# Autodesk Inventor assembly: Backhoe
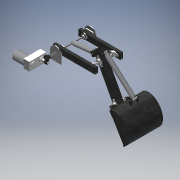
[picture p0: Inventor's stored thumbnail of the model, 180x180]
Saved by Autodesk Inventor 2019 (Build 230136000, 136)
## iProperties
Created: 2018-10-28
Part Number: Backhoe
Document SubType Name: Assembly
Designer: Alex Barnett
Mass: 10369.2 g
Surface Area: 11607 cm^2
Volume: 2447.16 cm^3
Density: 4.23725 g/cm^3
Author: Alex Barnett
## Documents named in this file (21)
- C:\Users\Alex Barnett\Documents\Machine Design\PR2\CAD\Backhoe.iam
- C:\Users\Alex Barnett\Documents\Machine Design\PR2\CAD\Boom Hinge.ipt
- C:\Users\Alex Barnett\Documents\Machine Design\PR2\CAD\Pin .5in. Dia. - Boom Hinge.ipt
- C:\Users\Alex Barnett\Documents\Machine Design\PR2\CAD\Steel 4130 1x2in. Tubing, t=.065in.,L=15in..ipt
- C:\Users\Alex Barnett\Documents\Machine Design\PR2\CAD\Steel 4130 1x2in. Tubing, t=.065in.,L=22in..ipt
- C:\Users\Alex Barnett\Documents\Machine Design\PR2\CAD\Boom to Stick .5in. Pin.ipt
- C:\Users\Alex Barnett\Documents\Machine Design\PR2\CAD\AmpFlow Motor & Gearbox.iam
- C:\Users\Alex Barnett\Documents\Machine Design\PR2\CAD\Worm Gear 12P 18T.ipt
- C:\Users\Alex Barnett\Documents\Machine Design\PR2\CAD\Steel 4130 1x2in. Tubing, t=.065in.,L=22in. Mirrored.ipt
- C:\Users\Alex Barnett\Documents\Machine Design\PR2\CAD\Stick to Scoop .5in. Pin.ipt
- C:\Users\Alex Barnett\Documents\Machine Design\PR2\CAD\Bucket.ipt
- C:\Users\Alex Barnett\Documents\Machine Design\PR2\CAD\Linear Actuator Top Pin .5in. Dia..ipt
- C:\Users\Alex Barnett\Documents\Machine Design\PR2\CAD\Linear Actuator Top Scoop Pin .5in. Dia..ipt
- C:\Users\Alex Barnett\Documents\Machine Design\PR2\CAD\Dry-Running Two-Bolt Flange Mounted Bearing, 0.5in. Diameter.ipt
- C:\Users\Alex Barnett\Documents\Machine Design\PR2\CAD\External Retaining Ring - Stainless Steel. 0.5in. Diameter.ipt
- C:\Users\Alex Barnett\Documents\Machine Design\PR2\CAD\Hub Connected to Steel Tubing - 0.5in. Diameter.ipt
- C:\Users\Alex Barnett\Documents\Machine Design\PR2\CAD\Tapered Roller Bearing Housing.ipt
- C:\Users\Alex Barnett\Documents\Machine Design\PR2\CAD\Tapered Roller Bearing, 0.5in. Diameter.ipt
- C:\Users\Alex Barnett\Documents\Machine Design\PR2\CAD\.125in. X .125in. Key, 1in. Long.ipt
- C:\Users\Alex Barnett\Documents\Machine Design\PR2\CAD\7.5 inch Linear Actuator.ipt
- C:\Users\Alex Barnett\Documents\Machine Design\PR2\CAD\9 inch Linear Actuator.ipt
## Components (45 placed, 20 different names)
1. Boom Hinge:1 — Mate:1, Mate:2, Mate:3, Flush:2, Mate:6, Mate:131, Mate:142, Mate:144, Mate:145, Mate:164
2. Boom Hinge:2 — Mate:5, Flush:2, Flush:5, Flush:11, Mate:129, Mate:147, Mate:149, Mate:150
3. Pin .5in. Dia. - Boom Hinge:1 — Mate:5, Mate:6, Flush:5, Mate:21, Mate:67, Mate:68, Mate:136, Mate:137, Mate:138, Mate:139, Mate:141, Mate:143, Mate:146, Mate:148, Mate:151, Mate:154, Flush:23, Mate:156, Mate:159, Mate:160, Mate:163, Mate:197
4. Steel 4130 1x2in. Tubing, t=.065in.,L=15in.:1 — Flush:6, Mate:21, Mate:110, Mate:112, Mate:113, Mate:130, Mate:131, Mate:140, Mate:152, Mate:158
5. Steel 4130 1x2in. Tubing, t=.065in.,L=15in.:2 — Flush:6, Mate:114, Mate:116, Mate:129, Mate:130, Mate:153, Mate:161, Mate:162, Mate:164
6. Boom to Stick .5in. Pin:1 — Mate:72, Mate:73, Mate:80, Mate:111, Mate:113, Mate:115, Mate:118, Mate:121, Mate:166, Mate:168, Mate:189, Mate:190, Mate:192
7. AmpFlow Motor & Gearbox:1 [sub-assembly] — Mate:69, Mate:70, Mate:71
8. Worm Gear 12P 18T:1 — Mate:67, Mate:68, Mate:69, Mate:70, Mate:71
9. Steel 4130 1x2in. Tubing, t=.065in.,L=22in.:1 — Mate:72, Mate:73, Flush:17, Mate:84, Mate:95, Mate:117, Mate:119, Mate:123, Mate:124, Mate:125, Mate:183, Mate:187
10. Steel 4130 1x2in. Tubing, t=.065in.,L=22in. Mirrored:1 — Mate:80, Flush:17, Mate:84, Flush:18, Mate:91, Flush:21, Flush:22, Mate:103, Mate:120, Mate:122, Mate:126, Mate:127, Mate:128, Mate:163, Mate:181, Mate:185
11. Stick to Scoop .5in. Pin:1 — Flush:18, Mate:169, Mate:170, Mate:174, Mate:176
12. Bucket:1 — Mate:170, Flush:24, Mate:171, Mate:172, Mate:173, Mate:175, Mate:177, Mate:179
13. Linear Actuator Top Pin .5in. Dia.:1 — Mate:91, Flush:21, Mate:182, Mate:184, Mate:199
14. Linear Actuator Top Scoop Pin .5in. Dia.:1 — Mate:171, Mate:172, Mate:178, Mate:180, Mate:200
15. Linear Actuator Top Pin .5in. Dia.:2 — Mate:95, Flush:22, Mate:186, Mate:188, Mate:198
16. Dry-Running Two-Bolt Flange Mounted Bearing, 0.5in. Diameter:5 — Mate:110, Mate:111, Mate:112, Mate:167
17. Dry-Running Two-Bolt Flange Mounted Bearing, 0.5in. Diameter:6 — Mate:114, Mate:115, Mate:116, Mate:165
18. Dry-Running Two-Bolt Flange Mounted Bearing, 0.5in. Diameter:7 — Mate:117, Mate:118, Mate:119, Mate:191
19. Dry-Running Two-Bolt Flange Mounted Bearing, 0.5in. Diameter:8 — Mate:120, Mate:121, Mate:122
20. Dry-Running Two-Bolt Flange Mounted Bearing, 0.5in. Diameter:9 — Mate:123, Mate:124, Mate:125, Mate:169
21. Dry-Running Two-Bolt Flange Mounted Bearing, 0.5in. Diameter:10 — Mate:126, Mate:127, Mate:128
22. External Retaining Ring - Stainless Steel. 0.5in. Diameter:1 — Mate:136, Mate:137
23. External Retaining Ring - Stainless Steel. 0.5in. Diameter:2 — Mate:138, Mate:139
24. Hub Connected to Steel Tubing - 0.5in. Diameter:1 — Mate:140, Mate:141, Mate:152, Flush:23, Mate:157
25. Tapered Roller Bearing Housing:1 — Mate:142, Mate:143, Mate:144
26. Tapered Roller Bearing, 0.5in. Diameter:1 — Mate:145, Mate:146
27. Tapered Roller Bearing Housing:2 — Mate:147, Mate:148, Mate:149
28. Tapered Roller Bearing, 0.5in. Diameter:2 — Mate:150, Mate:151
29. Hub Connected to Steel Tubing - 0.5in. Diameter:2 — Mate:153, Mate:154, Mate:161
30. .125in. X .125in. Key, 1in. Long:1 — Mate:156, Mate:157, Mate:158
31. .125in. X .125in. Key, 1in. Long:2 — Mate:159, Mate:160, Mate:162
32. External Retaining Ring - Stainless Steel. 0.5in. Diameter:3 — Mate:165, Mate:166
33. External Retaining Ring - Stainless Steel. 0.5in. Diameter:4 — Mate:167, Mate:168
34. External Retaining Ring - Stainless Steel. 0.5in. Diameter:5 — Mate:173, Mate:174
35. External Retaining Ring - Stainless Steel. 0.5in. Diameter:6 — Mate:175, Mate:176
36. External Retaining Ring - Stainless Steel. 0.5in. Diameter:7 — Mate:177, Mate:178
37. External Retaining Ring - Stainless Steel. 0.5in. Diameter:8 — Mate:179, Mate:180
38. External Retaining Ring - Stainless Steel. 0.5in. Diameter:9 — Mate:181, Mate:182
39. External Retaining Ring - Stainless Steel. 0.5in. Diameter:10 — Mate:183, Mate:184
40. External Retaining Ring - Stainless Steel. 0.5in. Diameter:11 — Mate:185, Mate:186
41. External Retaining Ring - Stainless Steel. 0.5in. Diameter:12 — Mate:187, Mate:188
42. External Retaining Ring - Stainless Steel. 0.5in. Diameter:13 — Mate:189, Mate:190
43. External Retaining Ring - Stainless Steel. 0.5in. Diameter:14 — Mate:191, Mate:192
44. 7.5 inch Linear Actuator:1 — Mate:197, Mate:198
45. 9 inch Linear Actuator:1 — Mate:199, Mate:200
## Relationships (112: Mate 100, Flush 12)
- Mate:1: Boom Hinge:1
- Mate:2: Boom Hinge:1
- Mate:3: Boom Hinge:1
- Mate:5: Boom Hinge:2 ↔ Pin .5in. Dia. - Boom Hinge:1
- Flush:2: Boom Hinge:1 ↔ Boom Hinge:2
- Mate:6: Boom Hinge:1 ↔ Pin .5in. Dia. - Boom Hinge:1
- Flush:5: Boom Hinge:2 ↔ Pin .5in. Dia. - Boom Hinge:1
- Flush:6: Steel 4130 1x2in. Tubing, t=.065in.,L=15in.:1 ↔ Steel 4130 1x2in. Tubing, t=.065in.,L=15in.:2
- Mate:21: Pin .5in. Dia. - Boom Hinge:1 ↔ Steel 4130 1x2in. Tubing, t=.065in.,L=15in.:1
- Flush:11: Boom Hinge:2
- Flush:12 (300 mm)
- Flush:13 (500 mm)
- Mate:67: Pin .5in. Dia. - Boom Hinge:1 ↔ Worm Gear 12P 18T:1
- Mate:68: Pin .5in. Dia. - Boom Hinge:1 ↔ Worm Gear 12P 18T:1
- Mate:69: AmpFlow Motor & Gearbox:1 ↔ Worm Gear 12P 18T:1
- Mate:70: AmpFlow Motor & Gearbox:1 ↔ Worm Gear 12P 18T:1
- Mate:71: AmpFlow Motor & Gearbox:1 ↔ Worm Gear 12P 18T:1
- Mate:72: Boom to Stick .5in. Pin:1 ↔ Steel 4130 1x2in. Tubing, t=.065in.,L=22in.:1
- Mate:73: Boom to Stick .5in. Pin:1 ↔ Steel 4130 1x2in. Tubing, t=.065in.,L=22in.:1
- Mate:80: Boom to Stick .5in. Pin:1 ↔ Steel 4130 1x2in. Tubing, t=.065in.,L=22in. Mirrored:1
- Flush:17: Steel 4130 1x2in. Tubing, t=.065in.,L=22in.:1 ↔ Steel 4130 1x2in. Tubing, t=.065in.,L=22in. Mirrored:1
- Mate:84: Steel 4130 1x2in. Tubing, t=.065in.,L=22in.:1 ↔ Steel 4130 1x2in. Tubing, t=.065in.,L=22in. Mirrored:1
- Flush:18: Steel 4130 1x2in. Tubing, t=.065in.,L=22in. Mirrored:1 ↔ Stick to Scoop .5in. Pin:1
- Mate:91: Steel 4130 1x2in. Tubing, t=.065in.,L=22in. Mirrored:1 ↔ Linear Actuator Top Pin .5in. Dia.:1
- Flush:21: Steel 4130 1x2in. Tubing, t=.065in.,L=22in. Mirrored:1 ↔ Linear Actuator Top Pin .5in. Dia.:1
- Mate:95: Steel 4130 1x2in. Tubing, t=.065in.,L=22in.:1 ↔ Linear Actuator Top Pin .5in. Dia.:2
- Flush:22: Steel 4130 1x2in. Tubing, t=.065in.,L=22in. Mirrored:1 ↔ Linear Actuator Top Pin .5in. Dia.:2
- Mate:103: Steel 4130 1x2in. Tubing, t=.065in.,L=22in. Mirrored:1
- Mate:110: Steel 4130 1x2in. Tubing, t=.065in.,L=15in.:1 ↔ Dry-Running Two-Bolt Flange Mounted Bearing, 0.5in. Diameter:5
- Mate:111: Boom to Stick .5in. Pin:1 ↔ Dry-Running Two-Bolt Flange Mounted Bearing, 0.5in. Diameter:5
- Mate:112: Steel 4130 1x2in. Tubing, t=.065in.,L=15in.:1 ↔ Dry-Running Two-Bolt Flange Mounted Bearing, 0.5in. Diameter:5
- Mate:113: Steel 4130 1x2in. Tubing, t=.065in.,L=15in.:1 ↔ Boom to Stick .5in. Pin:1
- Mate:114: Steel 4130 1x2in. Tubing, t=.065in.,L=15in.:2 ↔ Dry-Running Two-Bolt Flange Mounted Bearing, 0.5in. Diameter:6
- Mate:115: Boom to Stick .5in. Pin:1 ↔ Dry-Running Two-Bolt Flange Mounted Bearing, 0.5in. Diameter:6
- Mate:116: Steel 4130 1x2in. Tubing, t=.065in.,L=15in.:2 ↔ Dry-Running Two-Bolt Flange Mounted Bearing, 0.5in. Diameter:6
- Mate:117: Steel 4130 1x2in. Tubing, t=.065in.,L=22in.:1 ↔ Dry-Running Two-Bolt Flange Mounted Bearing, 0.5in. Diameter:7
- Mate:118: Boom to Stick .5in. Pin:1 ↔ Dry-Running Two-Bolt Flange Mounted Bearing, 0.5in. Diameter:7
- Mate:119: Steel 4130 1x2in. Tubing, t=.065in.,L=22in.:1 ↔ Dry-Running Two-Bolt Flange Mounted Bearing, 0.5in. Diameter:7
- Mate:120: Steel 4130 1x2in. Tubing, t=.065in.,L=22in. Mirrored:1 ↔ Dry-Running Two-Bolt Flange Mounted Bearing, 0.5in. Diameter:8
- Mate:121: Boom to Stick .5in. Pin:1 ↔ Dry-Running Two-Bolt Flange Mounted Bearing, 0.5in. Diameter:8
- Mate:122: Steel 4130 1x2in. Tubing, t=.065in.,L=22in. Mirrored:1 ↔ Dry-Running Two-Bolt Flange Mounted Bearing, 0.5in. Diameter:8
- Mate:123: Steel 4130 1x2in. Tubing, t=.065in.,L=22in.:1 ↔ Dry-Running Two-Bolt Flange Mounted Bearing, 0.5in. Diameter:9
- Mate:124: Steel 4130 1x2in. Tubing, t=.065in.,L=22in.:1 ↔ Dry-Running Two-Bolt Flange Mounted Bearing, 0.5in. Diameter:9
- Mate:125: Steel 4130 1x2in. Tubing, t=.065in.,L=22in.:1 ↔ Dry-Running Two-Bolt Flange Mounted Bearing, 0.5in. Diameter:9
- Mate:126: Steel 4130 1x2in. Tubing, t=.065in.,L=22in. Mirrored:1 ↔ Dry-Running Two-Bolt Flange Mounted Bearing, 0.5in. Diameter:10
- Mate:127: Steel 4130 1x2in. Tubing, t=.065in.,L=22in. Mirrored:1 ↔ Dry-Running Two-Bolt Flange Mounted Bearing, 0.5in. Diameter:10
- Mate:128: Steel 4130 1x2in. Tubing, t=.065in.,L=22in. Mirrored:1 ↔ Dry-Running Two-Bolt Flange Mounted Bearing, 0.5in. Diameter:10
- Mate:129 (25.4 mm): Boom Hinge:2 ↔ Steel 4130 1x2in. Tubing, t=.065in.,L=15in.:2
- Mate:130 (-254 mm): Steel 4130 1x2in. Tubing, t=.065in.,L=15in.:1 ↔ Steel 4130 1x2in. Tubing, t=.065in.,L=15in.:2
- Mate:131 (25.4 mm): Boom Hinge:1 ↔ Steel 4130 1x2in. Tubing, t=.065in.,L=15in.:1
- Mate:136: Pin .5in. Dia. - Boom Hinge:1 ↔ External Retaining Ring - Stainless Steel. 0.5in. Diameter:1
- Mate:137: Pin .5in. Dia. - Boom Hinge:1 ↔ External Retaining Ring - Stainless Steel. 0.5in. Diameter:1
- Mate:138: Pin .5in. Dia. - Boom Hinge:1 ↔ External Retaining Ring - Stainless Steel. 0.5in. Diameter:2
- Mate:139: Pin .5in. Dia. - Boom Hinge:1 ↔ External Retaining Ring - Stainless Steel. 0.5in. Diameter:2
- Mate:140: Steel 4130 1x2in. Tubing, t=.065in.,L=15in.:1 ↔ Hub Connected to Steel Tubing - 0.5in. Diameter:1
- Mate:141: Pin .5in. Dia. - Boom Hinge:1 ↔ Hub Connected to Steel Tubing - 0.5in. Diameter:1
- Mate:142: Boom Hinge:1 ↔ Tapered Roller Bearing Housing:1
- Mate:143: Pin .5in. Dia. - Boom Hinge:1 ↔ Tapered Roller Bearing Housing:1
- Mate:144: Boom Hinge:1 ↔ Tapered Roller Bearing Housing:1
- Mate:145: Boom Hinge:1 ↔ Tapered Roller Bearing, 0.5in. Diameter:1
- Mate:146: Pin .5in. Dia. - Boom Hinge:1 ↔ Tapered Roller Bearing, 0.5in. Diameter:1
- Mate:147: Boom Hinge:2 ↔ Tapered Roller Bearing Housing:2
- Mate:148: Pin .5in. Dia. - Boom Hinge:1 ↔ Tapered Roller Bearing Housing:2
- Mate:149: Boom Hinge:2 ↔ Tapered Roller Bearing Housing:2
- Mate:150: Boom Hinge:2 ↔ Tapered Roller Bearing, 0.5in. Diameter:2
- Mate:151: Pin .5in. Dia. - Boom Hinge:1 ↔ Tapered Roller Bearing, 0.5in. Diameter:2
- Mate:152: Steel 4130 1x2in. Tubing, t=.065in.,L=15in.:1 ↔ Hub Connected to Steel Tubing - 0.5in. Diameter:1
- Mate:153: Steel 4130 1x2in. Tubing, t=.065in.,L=15in.:2 ↔ Hub Connected to Steel Tubing - 0.5in. Diameter:2
- Mate:154: Pin .5in. Dia. - Boom Hinge:1 ↔ Hub Connected to Steel Tubing - 0.5in. Diameter:2
- Flush:23: Pin .5in. Dia. - Boom Hinge:1 ↔ Hub Connected to Steel Tubing - 0.5in. Diameter:1
- Mate:156: Pin .5in. Dia. - Boom Hinge:1 ↔ .125in. X .125in. Key, 1in. Long:1
- Mate:157: Hub Connected to Steel Tubing - 0.5in. Diameter:1 ↔ .125in. X .125in. Key, 1in. Long:1
- Mate:158: Steel 4130 1x2in. Tubing, t=.065in.,L=15in.:1 ↔ .125in. X .125in. Key, 1in. Long:1
- Mate:159: Pin .5in. Dia. - Boom Hinge:1 ↔ .125in. X .125in. Key, 1in. Long:2
- Mate:160: Pin .5in. Dia. - Boom Hinge:1 ↔ .125in. X .125in. Key, 1in. Long:2
- Mate:161: Steel 4130 1x2in. Tubing, t=.065in.,L=15in.:2 ↔ Hub Connected to Steel Tubing - 0.5in. Diameter:2
- Mate:162: Steel 4130 1x2in. Tubing, t=.065in.,L=15in.:2 ↔ .125in. X .125in. Key, 1in. Long:2
- Mate:163: Pin .5in. Dia. - Boom Hinge:1 ↔ Steel 4130 1x2in. Tubing, t=.065in.,L=22in. Mirrored:1
- Mate:164: Boom Hinge:1 ↔ Steel 4130 1x2in. Tubing, t=.065in.,L=15in.:2
- Mate:165: Dry-Running Two-Bolt Flange Mounted Bearing, 0.5in. Diameter:6 ↔ External Retaining Ring - Stainless Steel. 0.5in. Diameter:3
- Mate:166: Boom to Stick .5in. Pin:1 ↔ External Retaining Ring - Stainless Steel. 0.5in. Diameter:3
- Mate:167: Dry-Running Two-Bolt Flange Mounted Bearing, 0.5in. Diameter:5 ↔ External Retaining Ring - Stainless Steel. 0.5in. Diameter:4
- Mate:168: Boom to Stick .5in. Pin:1 ↔ External Retaining Ring - Stainless Steel. 0.5in. Diameter:4
- Mate:169: Stick to Scoop .5in. Pin:1 ↔ Dry-Running Two-Bolt Flange Mounted Bearing, 0.5in. Diameter:9
- Mate:170: Stick to Scoop .5in. Pin:1 ↔ Bucket:1
- Flush:24: Bucket:1
- Mate:171: Bucket:1 ↔ Linear Actuator Top Scoop Pin .5in. Dia.:1
- Mate:172: Bucket:1 ↔ Linear Actuator Top Scoop Pin .5in. Dia.:1
- Mate:173: Bucket:1 ↔ External Retaining Ring - Stainless Steel. 0.5in. Diameter:5
- Mate:174: Stick to Scoop .5in. Pin:1 ↔ External Retaining Ring - Stainless Steel. 0.5in. Diameter:5
- Mate:175: Bucket:1 ↔ External Retaining Ring - Stainless Steel. 0.5in. Diameter:6
- Mate:176: Stick to Scoop .5in. Pin:1 ↔ External Retaining Ring - Stainless Steel. 0.5in. Diameter:6
- Mate:177: Bucket:1 ↔ External Retaining Ring - Stainless Steel. 0.5in. Diameter:7
- Mate:178: Linear Actuator Top Scoop Pin .5in. Dia.:1 ↔ External Retaining Ring - Stainless Steel. 0.5in. Diameter:7
- Mate:179: Bucket:1 ↔ External Retaining Ring - Stainless Steel. 0.5in. Diameter:8
- Mate:180: Linear Actuator Top Scoop Pin .5in. Dia.:1 ↔ External Retaining Ring - Stainless Steel. 0.5in. Diameter:8
- Mate:181: Steel 4130 1x2in. Tubing, t=.065in.,L=22in. Mirrored:1 ↔ External Retaining Ring - Stainless Steel. 0.5in. Diameter:9
- Mate:182: Linear Actuator Top Pin .5in. Dia.:1 ↔ External Retaining Ring - Stainless Steel. 0.5in. Diameter:9
- Mate:183: Steel 4130 1x2in. Tubing, t=.065in.,L=22in.:1 ↔ External Retaining Ring - Stainless Steel. 0.5in. Diameter:10
- Mate:184: Linear Actuator Top Pin .5in. Dia.:1 ↔ External Retaining Ring - Stainless Steel. 0.5in. Diameter:10
- Mate:185: Steel 4130 1x2in. Tubing, t=.065in.,L=22in. Mirrored:1 ↔ External Retaining Ring - Stainless Steel. 0.5in. Diameter:11
- Mate:186: Linear Actuator Top Pin .5in. Dia.:2 ↔ External Retaining Ring - Stainless Steel. 0.5in. Diameter:11
- Mate:187: Steel 4130 1x2in. Tubing, t=.065in.,L=22in.:1 ↔ External Retaining Ring - Stainless Steel. 0.5in. Diameter:12
- Mate:188: Linear Actuator Top Pin .5in. Dia.:2 ↔ External Retaining Ring - Stainless Steel. 0.5in. Diameter:12
- Mate:189: Boom to Stick .5in. Pin:1 ↔ External Retaining Ring - Stainless Steel. 0.5in. Diameter:13
- Mate:190: Boom to Stick .5in. Pin:1 ↔ External Retaining Ring - Stainless Steel. 0.5in. Diameter:13
- Mate:191: Dry-Running Two-Bolt Flange Mounted Bearing, 0.5in. Diameter:7 ↔ External Retaining Ring - Stainless Steel. 0.5in. Diameter:14
- Mate:192: Boom to Stick .5in. Pin:1 ↔ External Retaining Ring - Stainless Steel. 0.5in. Diameter:14
- Mate:197: Pin .5in. Dia. - Boom Hinge:1 ↔ 7.5 inch Linear Actuator:1
- Mate:198: Linear Actuator Top Pin .5in. Dia.:2 ↔ 7.5 inch Linear Actuator:1
- Mate:199: Linear Actuator Top Pin .5in. Dia.:1 ↔ 9 inch Linear Actuator:1
- Mate:200: Linear Actuator Top Scoop Pin .5in. Dia.:1 ↔ 9 inch Linear Actuator:1
